# Autodesk Inventor assembly: GVS102
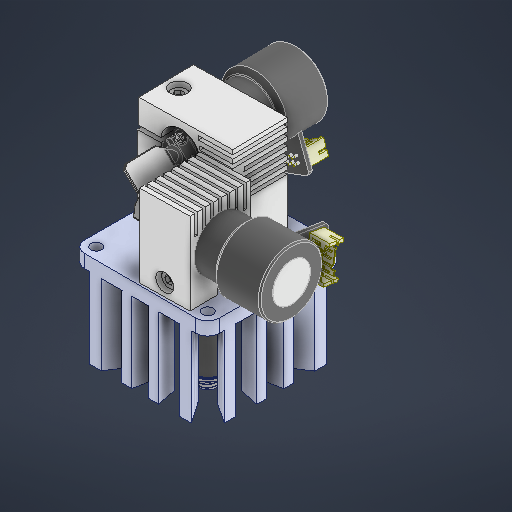
[picture p0: Inventor's stored thumbnail of the model, 512x512]
Saved by Autodesk Inventor 2025 (Build 290162000, 162)
## iProperties
Created: 2024-04-27
Part Number: GVS102
Document SubType Name: Assembly
Designer: Thienan Hoang
Author: Thienan Hoang
## Documents named in this file (7)
- C:\Users\mayhe\OneDrive\Documents\GitHub\In-situ-monitoring-of-powder-bed-fusion-additive-manufacturing\system_development\Orichalcum\v0.2\Hardware_design\galvo-scanner\GVS102.iam
- C:\Users\mayhe\OneDrive\Documents\GitHub\In-situ-monitoring-of-powder-bed-fusion-additive-manufacturing\system_development\Orichalcum\v0.2\Hardware_design\galvo-scanner\GHS003_M-Step.ipt
- C:\Users\mayhe\OneDrive\Documents\GitHub\In-situ-monitoring-of-powder-bed-fusion-additive-manufacturing\system_development\Orichalcum\v0.2\Hardware_design\galvo-scanner\GVS102-Step.ipt
- C:\Users\mayhe\OneDrive\Documents\GitHub\In-situ-monitoring-of-powder-bed-fusion-additive-manufacturing\system_development\Orichalcum\v0.2\Hardware_design\galvo-scanner\91292A110_18-8 Stainless Steel Socket Head Screw.ipt
- C:\Users\mayhe\OneDrive\Documents\GitHub\In-situ-monitoring-of-powder-bed-fusion-additive-manufacturing\system_development\Orichalcum\v0.2\Hardware_design\galvo-scanner\TRA30_M-Step.ipt
- C:\Users\mayhe\OneDrive\Documents\GitHub\In-situ-monitoring-of-powder-bed-fusion-additive-manufacturing\system_development\Orichalcum\v0.2\Hardware_design\galvo-scanner\TR1M-Step.ipt
- C:\Users\mayhe\OneDrive\Documents\GitHub\In-situ-monitoring-of-powder-bed-fusion-additive-manufacturing\system_development\Orichalcum\v0.2\Hardware_design\galvo-scanner\SS6MS12-Step.ipt
## Components (7 placed, 6 different names)
1. GVS102-Step:1 — Rotational:1
2. GHS003_M-Step:2 — Rotational:1, Mate:1, Mate:2, Rotational:2
3. 91292A110_18-8 Stainless Steel Socket Head Screw:1 — Mate:2
4. 91292A110_18-8 Stainless Steel Socket Head Screw:2 — Mate:1
5. TRA30_M-Step:1 — Rotational:2, Rotational:3, Mate:3
6. TR1M-Step:2 — Rotational:3, Mate:4
7. SS6MS12-Step:1 — Mate:3, Mate:4
## Relationships (8: Mate 4, RevoluteJoint 3, Flush 1)
- Rotational:1 [RevoluteJoint]: GVS102-Step:1 ↔ GHS003_M-Step:2
- Mate:1: GHS003_M-Step:2 ↔ 91292A110_18-8 Stainless Steel Socket Head Screw:2
- Mate:2: GHS003_M-Step:2 ↔ 91292A110_18-8 Stainless Steel Socket Head Screw:1
- Flush:1 (33.75 mm)
- Rotational:2 [RevoluteJoint]: GHS003_M-Step:2 ↔ TRA30_M-Step:1
- Rotational:3 [RevoluteJoint]: TRA30_M-Step:1 ↔ TR1M-Step:2
- Mate:3: TRA30_M-Step:1 ↔ SS6MS12-Step:1
- Mate:4 (5 mm): TR1M-Step:2 ↔ SS6MS12-Step:1
